# Autodesk Inventor assembly: outside_sleds
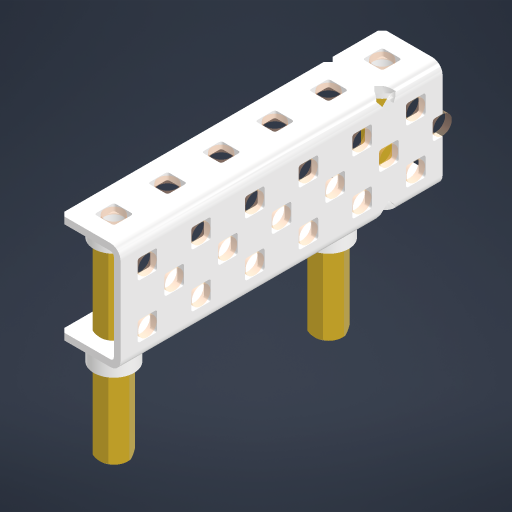
[picture p0: Inventor's stored thumbnail of the model, 512x512]
Saved by Autodesk Inventor 2023 (Build 270158000, 158)
## iProperties
Created: 2023-08-07
Part Number: outside_sleds
Document SubType Name: Assembly
Designer: srbel
Author: srbel
## Documents named in this file (6)
- C:\CAD\OverUnderCAD\Drive\outside_sleds.iam
- C:\CAD\OverUnderCAD\VEX-CAD-Inventor-1.4.0\Structure\C Channel\Aluminum 1x2x1\Alu C 1x2x1x6.ipt
- C:\CAD\OverUnderCAD\VEX-CAD-Inventor-1.4.0\Motion\Spacers\Spacer Nylon .313 OD\NSpacer .313 OD x .125.ipt
- C:\CAD\OverUnderCAD\VEX-CAD-Inventor-1.4.0\Motion\Spacers\Spacer Nylon .313 OD.ipt
- C:\CAD\OverUnderCAD\VEX-CAD-Inventor-1.4.0\Structure\Standoff\Standoff .75.ipt
- C:\CAD\OverUnderCAD\VEX-CAD-Inventor-1.4.0\Structure\Standoff.ipt
## Components (9 placed, 3 different names)
1. Alu C 1x2x1x6:1 — Insert:7
2. NSpacer .313 OD x .125:1
3. Standoff .75:1
4. NSpacer .313 OD x .125:2
5. Standoff .75:2
6. NSpacer .313 OD x .125:3
7. Standoff .75:3
8. NSpacer .313 OD x .125:4 — Insert:7, Insert:8
9. Standoff .75:4 — Insert:8
## Relationships (8: Insert 8)
- [Insert]: Alu C 1x2x1x6:1 ↔ NSpacer .313 OD x .125:1
- [Insert]: NSpacer .313 OD x .125:1 ↔ Standoff .75:1
- [Insert]: Alu C 1x2x1x6:1 ↔ NSpacer .313 OD x .125:2
- [Insert]: NSpacer .313 OD x .125:2 ↔ Standoff .75:2
- [Insert]: NSpacer .313 OD x .125:3 ↔ Standoff .75:3
- [Insert] (1.5875 mm): Alu C 1x2x1x6:1 ↔ NSpacer .313 OD x .125:3
- Insert:7 (1.5875 mm): Alu C 1x2x1x6:1 ↔ NSpacer .313 OD x .125:4
- Insert:8: NSpacer .313 OD x .125:4 ↔ Standoff .75:4
## Named parameters: d0_d4 = 0 mm, d1_d5 = 0 mm, d2_d6 = 0 mm, d3_d7 = 0 mm, d8_d5 = 0 mm
